# Autodesk Inventor assembly: Touch Segment
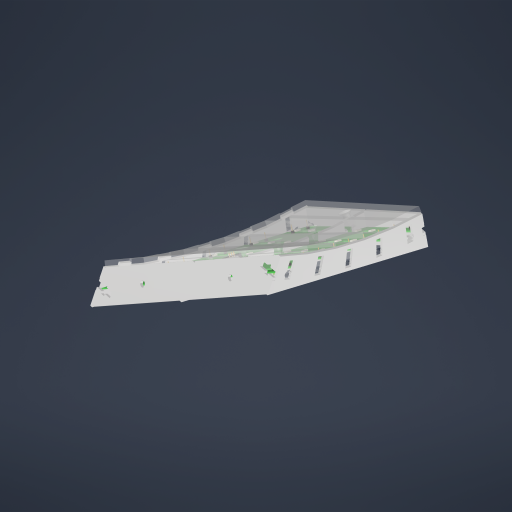
[picture p0: Inventor's stored thumbnail of the model, 512x512]
Saved by Autodesk Inventor 2023 (Build 270158000, 158)
## iProperties
Created: 2022-06-12
Part Number: Touch Segment
Document SubType Name: Assembly
Designer: FizzyApple12
Author: FizzyApple12
## Documents named in this file (10)
- C:\Users\FizzyApple12\Desktop\Wacca\WaccaController\Wacca Controller\Touch Segment\Touch Segment.iam
- C:\Users\FizzyApple12\Desktop\Wacca\WaccaController\Wacca Controller\Touch Segment\Touch Fifth.ipt
- C:\Users\FizzyApple12\Desktop\Wacca\WaccaController\Wacca Controller\Touch Segment\Back Plate.ipt
- C:\Users\FizzyApple12\Desktop\Wacca\WaccaController\Wacca Controller\Touch Segment\Front Plate.ipt
- C:\Users\FizzyApple12\Desktop\Wacca\WaccaController\Wacca Controller\Touch Segment\Center Plate.ipt
- C:\Users\FizzyApple12\Desktop\Wacca\WaccaController\Wacca Controller\Touch Segment\SidePlate.ipt
- C:\Users\FizzyApple12\Desktop\Wacca\WaccaController\Wacca Controller\Touch Segment\Joiner.ipt
- C:\Users\FizzyApple12\Desktop\Wacca\WaccaController\Wacca Controller\Touch Segment\Inner Bracket.ipt
- C:\Users\FizzyApple12\Desktop\Wacca\WaccaController\Wacca Controller\Touch Segment\PCB.ipt
- C:\Users\FizzyApple12\Desktop\Wacca\WaccaController\Wacca Controller\WaccaTouchPanel-pcb.ipt
## Components (19 placed, 9 different names)
1. Touch Fifth:1 — Mate:1, Mate:5, Flush:1, Mate:19
2. Touch Fifth:2 — Mate:1, Mate:2, Mate:5, Mate:6
3. Touch Fifth:3 — Mate:2, Mate:3, Mate:6, Mate:7, Mate:8, Flush:2, Mate:11, Flush:3, Mate:12, Flush:10
4. Touch Fifth:4 — Mate:3, Mate:4, Mate:7
5. Touch Fifth:5 — Mate:4, Mate:8, Flush:4, Mate:17, Mate:18
6. Back Plate:1 — Flush:1, Mate:23, Mate:24, Mate:25
7. Front Plate:1 — Flush:2, Mate:11, Flush:6, Flush:7, Flush:8, Flush:9, Mate:26, Mate:27, Mate:28, Mate:29, Mate:30, Mate:31, Mate:32, Mate:33, Mate:34, Mate:35, Mate:36, Mate:37, Mate:38
8. Center Plate:1 — Flush:3, Mate:12, Flush:4
9. SidePlate:1
10. SidePlate:2
11. Joiner:1 — Flush:6, Flush:7
12. Joiner:2 — Mate:23, Mate:24, Mate:25
13. Inner Bracket:1 — Flush:8, Flush:9, Mate:28
14. Inner Bracket:2 — Mate:30, Mate:31, Mate:32
15. Inner Bracket:3 — Mate:29, Mate:33, Mate:34
16. Inner Bracket:4 — Mate:27, Mate:35, Mate:36
17. Inner Bracket:5 — Mate:26, Mate:37, Mate:38
18. PCB:1 — Flush:11, Flush:12, Mate:39, Mate:40
19. WaccaTouchPanel-pcb:1 — Mate:39, Mate:40
## Relationships (49: Mate 37, Flush 12)
- Mate:1: Touch Fifth:1 ↔ Touch Fifth:2
- Mate:2: Touch Fifth:2 ↔ Touch Fifth:3
- Mate:3: Touch Fifth:3 ↔ Touch Fifth:4
- Mate:4: Touch Fifth:4 ↔ Touch Fifth:5
- Mate:5: Touch Fifth:1 ↔ Touch Fifth:2
- Mate:6: Touch Fifth:2 ↔ Touch Fifth:3
- Mate:7: Touch Fifth:3 ↔ Touch Fifth:4
- Mate:8: Touch Fifth:3 ↔ Touch Fifth:5
- Flush:1: Touch Fifth:1 ↔ Back Plate:1
- Flush:2: Touch Fifth:3 ↔ Front Plate:1
- Mate:11: Touch Fifth:3 ↔ Front Plate:1
- Flush:3: Touch Fifth:3 ↔ Center Plate:1
- Mate:12: Touch Fifth:3 ↔ Center Plate:1
- Flush:4: Touch Fifth:5 ↔ Center Plate:1
- [Flush]: Center Plate:1 ↔ SidePlate:1
- [Mate]: Touch Fifth:1 ↔ SidePlate:1
- [Mate]: Touch Fifth:1 ↔ SidePlate:1
- [Mate]: Touch Fifth:5 ↔ SidePlate:1
- Mate:17: Touch Fifth:5
- Mate:18: Touch Fifth:5
- Mate:19: Touch Fifth:1
- [Mate]: Front Plate:1 ↔ SidePlate:2
- [Mate]: SidePlate:2
- [Mate]: Touch Fifth:5 ↔ SidePlate:2
- Flush:6: Front Plate:1 ↔ Joiner:1
- Flush:7: Front Plate:1 ↔ Joiner:1
- Mate:23: Back Plate:1 ↔ Joiner:2
- Mate:24: Back Plate:1 ↔ Joiner:2
- Mate:25: Back Plate:1 ↔ Joiner:2
- Flush:8: Front Plate:1 ↔ Inner Bracket:1
- Flush:9: Front Plate:1 ↔ Inner Bracket:1
- Mate:26: Front Plate:1 ↔ Inner Bracket:5
- Mate:27: Front Plate:1 ↔ Inner Bracket:4
- Mate:28: Front Plate:1 ↔ Inner Bracket:1
- Mate:29: Front Plate:1 ↔ Inner Bracket:3
- Mate:30: Front Plate:1 ↔ Inner Bracket:2
- Mate:31: Front Plate:1 ↔ Inner Bracket:2
- Mate:32: Front Plate:1 ↔ Inner Bracket:2
- Mate:33: Front Plate:1 ↔ Inner Bracket:3
- Mate:34: Front Plate:1 ↔ Inner Bracket:3
- Mate:35: Front Plate:1 ↔ Inner Bracket:4
- Mate:36: Front Plate:1 ↔ Inner Bracket:4
- Mate:37: Front Plate:1 ↔ Inner Bracket:5
- Mate:38: Front Plate:1 ↔ Inner Bracket:5
- Flush:10 (-12.7 mm): Touch Fifth:3
- Flush:11: PCB:1
- Flush:12: PCB:1
- Mate:39: PCB:1 ↔ WaccaTouchPanel-pcb:1
- Mate:40: PCB:1 ↔ WaccaTouchPanel-pcb:1
